# Autodesk Inventor assembly: Intake
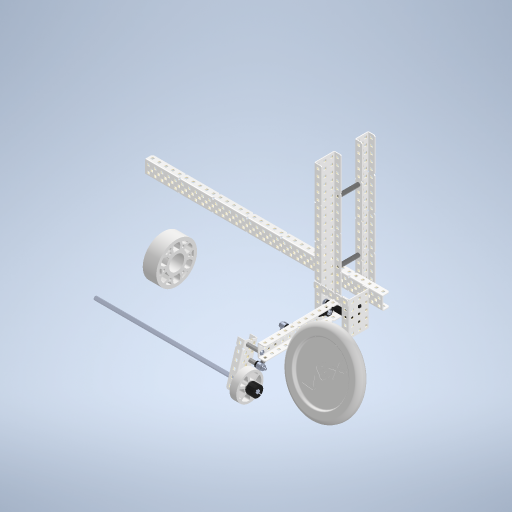
[picture p0: Inventor's stored thumbnail of the model, 512x512]
Saved by Autodesk Inventor 2023 (Build 270158000, 158)
## iProperties
Created: 2022-09-02
Part Number: Intake
Document SubType Name: Assembly
Designer: alex
Author: alex
## Documents named in this file (35)
- C:\Users\alex\Documents\GitHub\4067X_spin_up_cad\Mechanism\Intake.iam
- C:\Users\alex\Documents\GitHub\4067X_spin_up_cad\Library\Structure\Standoff\Standoff 1.00.ipt
- C:\Users\alex\Documents\GitHub\4067X_spin_up_cad\Library\Structure\Standoff.ipt
- C:\Users\alex\Documents\GitHub\4067X_spin_up_cad\Library\Structure\Standoff\Standoff 2.00.ipt
- C:\Users\alex\Documents\GitHub\4067X_spin_up_cad\Library\Structure\Hardware\Screw Steel - Star\SScrew Star Smooth .290.ipt
- C:\Users\alex\Documents\GitHub\4067X_spin_up_cad\Library\Structure\Hardware\Screw Steel - Star.ipt
- C:\Users\alex\Documents\GitHub\4067X_spin_up_cad\Library\Structure\Standoff\Standoff .50.ipt
- C:\Users\alex\Documents\GitHub\4067X_spin_up_cad\Library\Motion\Spacers\Spacer Nylon .375 OD.ipt
- C:\Users\alex\Documents\GitHub\4067X_spin_up_cad\Library\Structure\C-Channels\Aluminum 1x2x1\Alu C 1x2x1x6.ipt
- C:\Users\alex\Documents\GitHub\4067X_spin_up_cad\Library\Motion\Shaft HS\Shaft HS\Shaft HS 12.0 in.ipt
- C:\Users\alex\Documents\GitHub\4067X_spin_up_cad\Library\Motion\Shaft HS\Shaft HS.ipt
- C:\Users\alex\Documents\GitHub\4067X_spin_up_cad\Library\Motion\Spacers\Spacer Nylon .375 OD\NSpacer .375 OD x .125.ipt
- C:\Users\alex\Documents\GitHub\4067X_spin_up_cad\Library\Motion\Shaft Collar with Set Screw.ipt
- C:\Users\alex\Documents\GitHub\4067X_spin_up_cad\WithAdapter2Inch.iam
- C:\Users\alex\Documents\GitHub\4067X_spin_up_cad\Library\Motion\Shaft HS\HS Shaft Collar.ipt
- C:\Users\alex\Documents\GitHub\4067X_spin_up_cad\Library\Structure\Hardware\Screw Steel - Star\SScrew Star Smooth 1.250.ipt
- C:\Users\alex\Documents\GitHub\4067X_spin_up_cad\Library\Structure\Hardware\Nut Keps.ipt
- C:\Users\alex\Documents\GitHub\4067X_spin_up_cad\Library\Structure\Hardware\Screw Steel - Star\SScrew Star Smooth .625.ipt
- C:\Users\alex\Documents\GitHub\4067X_spin_up_cad\Library\Structure\C-Channels\Aluminum 1x2x1\Alu C 1x2x1x12.ipt
- C:\Users\alex\Documents\GitHub\4067X_spin_up_cad\Library\Motion\1-Post Bearing Flat Hex Retainer.ipt
- C:\Users\alex\Documents\GitHub\4067X_spin_up_cad\Library\Structure\Hardware\Screw Steel - Star\SScrew Star Smooth .375.ipt
- C:\Users\alex\Documents\GitHub\4067X_spin_up_cad\Library\Structure\Hardware\Nut Nylock.ipt
- C:\Users\alex\Documents\GitHub\4067X_spin_up_cad\Library\Structure\C-Channels\Aluminum 1x3x1\Alu C 1x3x1x20.ipt
- C:\Users\alex\Documents\GitHub\4067X_spin_up_cad\SpinUp\Disc.iam
- C:\Users\alex\Documents\GitHub\4067X_spin_up_cad\Library\Structure\C-Channels\Aluminum 1x3x1\Alu C 1x3x1x5.ipt
- C:\Users\alex\Documents\GitHub\4067X_spin_up_cad\Library\Structure\C-Channels\Aluminum 1x2x1\Alu C 1x2x1x35.ipt
- C:\Users\alex\Documents\GitHub\4067X_spin_up_cad\Library\Structure\C-Channels\Aluminum 1x2x1\Alu C 1x2x1x20.ipt
- C:\Users\alex\Documents\GitHub\4067X_spin_up_cad\Library\Structure\Plates\Aluminum\VEX Plates\Alu Plate VEX 1x5.ipt
- C:\Users\alex\Documents\GitHub\4067X_spin_up_cad\Library\Structure\Hardware\Screw Steel - Star\SScrew Star Smooth 2.500.ipt
- C:\Users\alex\Documents\GitHub\4067X_spin_up_cad\Library\Motion\Spacers\Spacer Nylon .375 OD\NSpacer .375 OD x .375.ipt
- C:\Users\alex\Documents\GitHub\4067X_spin_up_cad\Library\Motion\Spacers\Washer Steel\SWasher .375 OD x .015625.ipt
- C:\Users\alex\Documents\GitHub\4067X_spin_up_cad\Library\Motion\Spacers\Washer Steel.ipt
- C:\Users\alex\Documents\GitHub\4067X_spin_up_cad\Library\Motion\Spacers\Spacer Nylon .375 OD\NSpacer .375 OD x .500.ipt
- C:\Users\alex\Documents\GitHub\4067X_spin_up_cad\Library\Motion\Wheels\Flex Wheels\3.000 Flex Wheel\3.000 30A 1.000.ipt
- C:\Users\alex\Documents\GitHub\4067X_spin_up_cad\Library\Motion\Wheels\Flex Wheels\3.000 Flex Wheel.ipt
## Components (40 placed, 28 different names)
1. Alu C 1x2x1x6:1 — Mate:2, Mate:3, Insert:39, Insert:40, Mate:11, Insert:48, Insert:50
2. Shaft HS 12.0 in:1 — Mate:2, Mate:5, Mate:6, Mate:9, Mate:10, Flush:1
3. NSpacer .375 OD x .125:1 — Insert:34, Insert:73
4. Shaft Collar with Set Screw:1 — Insert:34, Mate:4, Mate:7, Insert:53
5. Shaft Collar with Set Screw:2 — Mate:3, Mate:4, Insert:35, Insert:49
6. WithAdapter2Inch:1 [sub-assembly] — Mate:5, Mate:6, Mate:8, Mate:11
7. Standoff 2.00:12 — Insert:35, Mate:7
8. Standoff .50:14 — Insert:38, Insert:39
9. NSpacer .375 OD x .125:2 — Insert:38
10. Standoff 1.00:15 — Insert:40, Insert:71
11. HS Shaft Collar:1 — Mate:8, Mate:9, Mate:10, Flush:1
12. SScrew Star Smooth 1.250:13 — Insert:48
13. Nut Keps:1 — Insert:49
14. SScrew Star Smooth .290:14 — Insert:50
15. SScrew Star Smooth .290:15 — Insert:72
16. SScrew Star Smooth .625:16 — Insert:74
17. Nut Keps:2 — Insert:53
18. Alu C 1x2x1x12:1 — Insert:71, Insert:72, Insert:73, Insert:74, Insert:102, Mate:12, Insert:103, Mate:14
19. 1-Post Bearing Flat Hex Retainer:1 — Insert:102, Mate:12, Insert:104, Mate:13, Insert:121
20. SScrew Star Smooth .375:30 — Insert:103
21. Nut Nylock:1 — Insert:104
22. Alu C 1x3x1x20:1 — Mate:13, Mate:14, Insert:105, Insert:106, Insert:109, Insert:113, Insert:115, Insert:116, Insert:117
23. Alu C 1x3x1x5:1 — Insert:107, Insert:108, Insert:114, Insert:120, Mate:15
24. Alu C 1x2x1x35:1 — Insert:105, Insert:106, Insert:107, Insert:108
25. Alu C 1x2x1x20:1 — Insert:111
26. Standoff 1.00:16 — Insert:109, Insert:110
27. Standoff .50:17 — Insert:110, Insert:111
28. Standoff 1.00:18 — Insert:113
29. Standoff .50:19
30. Alu Plate VEX 1x5:1 — Insert:114, Insert:115
31. SScrew Star Smooth 2.500:31 — Insert:116
32. Nut Keps:3 — Insert:117, Insert:118
33. NSpacer .375 OD x .375:3 — Insert:119
34. SWasher .375 OD x .015625:1 — Insert:118, Insert:119
35. 1-Post Bearing Flat Hex Retainer:2 — Insert:120, Mate:15
36. NSpacer .375 OD x .500:4 — Insert:121, Insert:122
37. NSpacer .375 OD x .500:5 — Insert:122, Insert:123
38. NSpacer .375 OD x .375:6 — Insert:123
39. Disc:1 [sub-assembly]
40. 3.000 30A 1.000:1
## Relationships (50: Insert 35, Mate 14, Flush 1)
- Mate:2: Alu C 1x2x1x6:1 ↔ Shaft HS 12.0 in:1
- Insert:34: NSpacer .375 OD x .125:1 ↔ Shaft Collar with Set Screw:1
- Mate:3: Alu C 1x2x1x6:1 ↔ Shaft Collar with Set Screw:2
- Mate:4: Shaft Collar with Set Screw:1 ↔ Shaft Collar with Set Screw:2
- Mate:5: Shaft HS 12.0 in:1 ↔ WithAdapter2Inch:1
- Mate:6: Shaft HS 12.0 in:1 ↔ WithAdapter2Inch:1
- Insert:35 (-0.3556 mm): Shaft Collar with Set Screw:2 ↔ Standoff 2.00:12
- Mate:7 (-0.3556 mm): Shaft Collar with Set Screw:1 ↔ Standoff 2.00:12
- Insert:38: Standoff .50:14 ↔ NSpacer .375 OD x .125:2
- Insert:39: Alu C 1x2x1x6:1 ↔ Standoff .50:14
- Insert:40: Alu C 1x2x1x6:1 ↔ Standoff 1.00:15
- Mate:8: WithAdapter2Inch:1 ↔ HS Shaft Collar:1
- Mate:9: Shaft HS 12.0 in:1 ↔ HS Shaft Collar:1
- Mate:10: Shaft HS 12.0 in:1 ↔ HS Shaft Collar:1
- Flush:1 (-0.3556 mm): Shaft HS 12.0 in:1 ↔ HS Shaft Collar:1
- Mate:11: Alu C 1x2x1x6:1 ↔ WithAdapter2Inch:1
- Insert:48: Alu C 1x2x1x6:1 ↔ SScrew Star Smooth 1.250:13
- Insert:49: Shaft Collar with Set Screw:2 ↔ Nut Keps:1
- Insert:50: Alu C 1x2x1x6:1 ↔ SScrew Star Smooth .290:14
- Insert:53: Shaft Collar with Set Screw:1 ↔ Nut Keps:2
- Insert:71: Standoff 1.00:15 ↔ Alu C 1x2x1x12:1
- Insert:72: SScrew Star Smooth .290:15 ↔ Alu C 1x2x1x12:1
- Insert:73: NSpacer .375 OD x .125:1 ↔ Alu C 1x2x1x12:1
- Insert:74: SScrew Star Smooth .625:16 ↔ Alu C 1x2x1x12:1
- Insert:102: Alu C 1x2x1x12:1 ↔ 1-Post Bearing Flat Hex Retainer:1
- Mate:12: Alu C 1x2x1x12:1 ↔ 1-Post Bearing Flat Hex Retainer:1
- Insert:103: Alu C 1x2x1x12:1 ↔ SScrew Star Smooth .375:30
- Insert:104: 1-Post Bearing Flat Hex Retainer:1 ↔ Nut Nylock:1
- Mate:13: 1-Post Bearing Flat Hex Retainer:1 ↔ Alu C 1x3x1x20:1
- Mate:14 (13.6398 mm): Alu C 1x2x1x12:1 ↔ Alu C 1x3x1x20:1
- Insert:105: Alu C 1x3x1x20:1 ↔ Alu C 1x2x1x35:1
- Insert:106: Alu C 1x3x1x20:1 ↔ Alu C 1x2x1x35:1
- Insert:107: Alu C 1x3x1x5:1 ↔ Alu C 1x2x1x35:1
- Insert:108: Alu C 1x3x1x5:1 ↔ Alu C 1x2x1x35:1
- Insert:109: Alu C 1x3x1x20:1 ↔ Standoff 1.00:16
- Insert:110: Standoff 1.00:16 ↔ Standoff .50:17
- Insert:111: Alu C 1x2x1x20:1 ↔ Standoff .50:17
- [Insert]: Standoff 1.00:18 ↔ Standoff .50:19
- Insert:113: Alu C 1x3x1x20:1 ↔ Standoff 1.00:18
- Insert:114: Alu C 1x3x1x5:1 ↔ Alu Plate VEX 1x5:1
- Insert:115: Alu C 1x3x1x20:1 ↔ Alu Plate VEX 1x5:1
- Insert:116: Alu C 1x3x1x20:1 ↔ SScrew Star Smooth 2.500:31
- Insert:117: Alu C 1x3x1x20:1 ↔ Nut Keps:3
- Insert:118: Nut Keps:3 ↔ SWasher .375 OD x .015625:1
- Insert:119: NSpacer .375 OD x .375:3 ↔ SWasher .375 OD x .015625:1
- Insert:120: Alu C 1x3x1x5:1 ↔ 1-Post Bearing Flat Hex Retainer:2
- Mate:15: Alu C 1x3x1x5:1 ↔ 1-Post Bearing Flat Hex Retainer:2
- Insert:121: 1-Post Bearing Flat Hex Retainer:1 ↔ NSpacer .375 OD x .500:4
- Insert:122: NSpacer .375 OD x .500:4 ↔ NSpacer .375 OD x .500:5
- Insert:123: NSpacer .375 OD x .500:5 ↔ NSpacer .375 OD x .375:6
## Named parameters: d171_d169 = 0 mm
